# Autodesk Inventor assembly: 3in flex wheel holder assembly
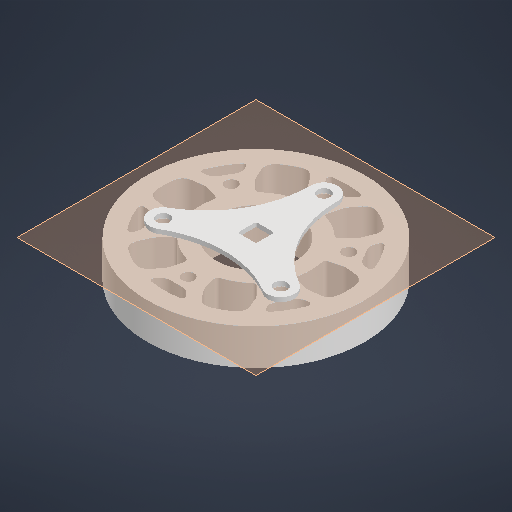
[picture p0: Inventor's stored thumbnail of the model, 512x512]
Saved by Autodesk Inventor 2025.4 (Build 294407000, 407)
## iProperties
Created: 2026-01-22
Part Number: 3in flex wheel holder assembly
Document SubType Name: Assembly
Designer: shaun
Author: shaun
## Documents named in this file (4)
- C:\Users\shaun\Documents\AURA Pushback Github\aura-cad\15\3in flex wheel holder assembly.iam
- C:\Users\shaun\Documents\AURA Pushback Github\aura-cad\!lib\Motion\Wheels\Flex Wheels\3.000 Flex Wheel\3.000 30A .500.ipt
- C:\Users\shaun\Documents\AURA Pushback Github\aura-cad\!lib\Motion\Wheels\Flex Wheels\3.000 Flex Wheel.ipt
- C:\Users\shaun\Documents\AURA Pushback Github\aura-cad\15\3in flex wheel holder.ipt
## Components (2 placed, 2 different names)
1. 3.000 30A .500:1 — Flush:1, Flush:2
2. 3in flex wheel holder:1 — Flush:1, Flush:2
## Relationships (2: Flush 2)
- Flush:1: 3.000 30A .500:1 ↔ 3in flex wheel holder:1
- Flush:2: 3.000 30A .500:1 ↔ 3in flex wheel holder:1
